# Autodesk Inventor assembly: HHPFRN5
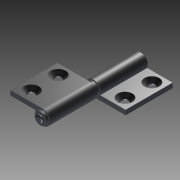
[picture p0: Inventor's stored thumbnail of the model, 180x180]
Saved by Autodesk Inventor 2015 SP1 (Build 190203100, 203)
## iProperties
Category: PARTsolutions
Company: MISUMI
Created: 2015-01-26
Part Number: HHPFRN5
Catalog Web Link: www.cadenas.de
Description: HHPFLN, HHPFRN-Aluminum Flag Hinges
Vendor: MISUMI
Document SubType Name: Assembly
Designer: PARTuser1
Manufacturer: MISUMI
PSOL_IDENT_0: {\\10.0.0.236\data_v8\23d-libs\misumi\metric\39_accessories_for_al_extrusions\hhpfln_asmtab.prj},176
PSOL_IDENT_1: {VTYP=3D},{STYP=ASSTAB},{NB=HHPFRN5},{LINA=HHPFRN5},{NN=HHPFLN, HHPFRN},{DATE=17.11.2014 05:31:02},
PSOL_IDENT_2: {GEOMDATE=07.05.2009},{VERSION=},{LINEID=10},{LINESUBID=-1},{WBVAR=TS,ALT1}  {NB=HHPFRN5},{LINA=HHPF
PSOL_IDENT_3: RN5},{KT=DUMMY},{PN=HHPFRN5},{TYPE=HHPFRN},{TS=HHPFRN},{MAT=6063 Aluminum Bushing - Polyacetal},{ST=
PSOL_IDENT_4: Anodizing},{NO=5},{ALKG=10},{ALN=98},{MASS=36},{L=35},{W=48},{K=7.5},{P=20},{J=8.0},{F=16.0},{V=10.5
PSOL_IDENT_5: },{ND=5.5},{NC=11},{T=3.5},{Y=38.5},{AB=FB5-8},{QB=4},{AN=HNTT5-5},{QN=4},{ALT1=},{PPATH=hhpfln_temp
PSOL_IDENT_6: l.prj}
SUPPLIER: MISUMI
ARTICLENO: HHPFRN5
BOMINFO: HHPFRN5
CREATOR: CADENAS GmbH
Title: HHPFRN5
Author: Cadenas PARTsolutions
Comments: Aluminum Flag Hinges
## Documents named in this file (3)
- C:\Users\Jack\ownCloud\Projects\CoreXY\InventorModel\Hardware\Hinges\HingeHHPFRN5\HHPFRN5.iam
- C:\Users\Jack\ownCloud\Projects\CoreXY\InventorModel\Hardware\Hinges\HingeHHPFRN5\HHPFRN5_1.ipt
- C:\Users\Jack\ownCloud\Projects\CoreXY\InventorModel\Hardware\Hinges\HingeHHPFRN5\HHPFRN5_2.ipt
## Components (2 placed, 2 different names)
1. HHPFRN5_1:1 — Mate:1, Flush:1
2. HHPFRN5_2:1 — Mate:1, Flush:1
## Relationships (2: Mate 1, Flush 1)
- Mate:1: HHPFRN5_1:1 ↔ HHPFRN5_2:1
- Flush:1: HHPFRN5_1:1 ↔ HHPFRN5_2:1
